# Autodesk Inventor assembly: Shooter assembly
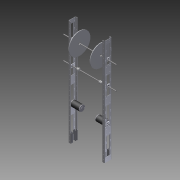
[picture p0: Inventor's stored thumbnail of the model, 180x180]
Saved by Autodesk Inventor 2014 SP1 (Build 180222100, 222)
## iProperties
Created: 2014-02-21
Part Number: Shooter assembly
Document SubType Name: Assembly
Designer: Asif
Author: Asif
## Documents named in this file (9)
- C:\Users\Asif\Documents\GitHub\CAD\CAD Team 2014\Shooter\Shooter assembly.iam
- C:\Users\Asif\Documents\GitHub\CAD\CAD Team 2014\Shooter\U-CHANNEL 6 Sot_sheet metal Edited to size.ipt
- C:\Users\Asif\Documents\GitHub\CAD\CAD Team 2014\Shooter\8020-1010 edited to size.ipt
- C:\Users\Asif\Documents\GitHub\CAD\CAD Team 2014\Shooter\CIM RECEIVER - AM-0860.ipt
- C:\Users\Asif\Documents\GitHub\CAD\CAD Team 2014\Shooter\3-8 bearing.ipt
- C:\Users\Asif\Documents\GitHub\CAD\CAD Team 2014\Shooter\80t Sprocket.ipt
- C:\Users\Asif\Documents\GitHub\CAD\CAD Team 2014\Shooter\3-8 Shooter Shaft.ipt
- C:\Users\Asif\Documents\GitHub\CAD\CAD Team 2014\Shooter\10 th sprocket.ipt
- C:\Users\Asif\Documents\GitHub\CAD\CAD Team 2014\Shooter\CIM motor.ipt
## Components (24 placed, 8 different names)
1. U-CHANNEL 6 Sot_sheet metal Edited to size:1 — Mate:1, Mate:2, Mate:3, Mate:4, Flush:2, Flush:5, Flush:6, Flush:7, Mate:16, Mate:17, Mate:25, Mate:26, Flush:13, Mate:27, Mate:28
2. U-CHANNEL 6 Sot_sheet metal Edited to size:2 — Mate:5, Mate:6, Flush:3, Mate:7, Mate:8, Flush:4, Flush:6, Flush:7, Mate:10, Mate:11, Mate:12, Mate:13, Mate:14, Mate:15, Flush:13
3. 8020-1010 edited to size:1 — Mate:3, Mate:4, Flush:2
4. 8020-1010 edited to size:2 — Mate:1, Mate:2, Flush:5, Tangent:1
5. 8020-1010 edited to size:3 — Mate:5, Mate:6, Flush:3, Tangent:1
6. 8020-1010 edited to size:4 — Mate:7, Mate:8, Flush:4
7. CIM RECEIVER - AM-0860:1 — Insert:8, Flush:9, Mate:25, Mate:26
8. CIM RECEIVER - AM-0860:2 — Mate:14, Mate:15, Insert:4, Flush:8
9. CIM RECEIVER - AM-0860:3 — Mate:10, Mate:11, Insert:7, Flush:9
10. CIM RECEIVER - AM-0860:4 — Mate:12, Mate:13, Flush:10, Insert:14
11. CIM RECEIVER - AM-0860:5 — Flush:10, Insert:13, Mate:27, Mate:28
12. CIM RECEIVER - AM-0860:6 — Mate:16, Mate:17, Insert:1, Flush:8
13. 3-8 bearing:2 — Insert:4, Mate:22, Insert:12
14. 3-8 bearing:3 — Insert:7
15. 3-8 bearing:4 — Insert:1, Mate:21, Insert:9, Insert:11
16. 3-8 bearing:6 — Insert:8, Insert:10
17. 80t Sprocket:1 — Insert:11, Flush:11
18. 80t Sprocket:2 — Insert:12, Flush:12
19. 3-8 Shooter Shaft:1 — Insert:9
20. 3-8 Shooter Shaft:2 — Insert:10, Mate:23, Mate:24
21. 10 th sprocket:1 — Flush:11, Mate:23
22. 10 th sprocket:2 — Flush:12, Mate:24
23. CIM motor:1 — Insert:13
24. CIM motor:2 — Insert:14
## Relationships (47: Mate 24, Flush 12, Insert 10, Tangent 1)
- Mate:1: U-CHANNEL 6 Sot_sheet metal Edited to size:1 ↔ 8020-1010 edited to size:2
- Mate:2: U-CHANNEL 6 Sot_sheet metal Edited to size:1 ↔ 8020-1010 edited to size:2
- Mate:3: U-CHANNEL 6 Sot_sheet metal Edited to size:1 ↔ 8020-1010 edited to size:1
- Mate:4: U-CHANNEL 6 Sot_sheet metal Edited to size:1 ↔ 8020-1010 edited to size:1
- Flush:2: U-CHANNEL 6 Sot_sheet metal Edited to size:1 ↔ 8020-1010 edited to size:1
- Mate:5: U-CHANNEL 6 Sot_sheet metal Edited to size:2 ↔ 8020-1010 edited to size:3
- Mate:6: U-CHANNEL 6 Sot_sheet metal Edited to size:2 ↔ 8020-1010 edited to size:3
- Flush:3: U-CHANNEL 6 Sot_sheet metal Edited to size:2 ↔ 8020-1010 edited to size:3
- Mate:7: U-CHANNEL 6 Sot_sheet metal Edited to size:2 ↔ 8020-1010 edited to size:4
- Mate:8: U-CHANNEL 6 Sot_sheet metal Edited to size:2 ↔ 8020-1010 edited to size:4
- Flush:4: U-CHANNEL 6 Sot_sheet metal Edited to size:2 ↔ 8020-1010 edited to size:4
- Flush:5: U-CHANNEL 6 Sot_sheet metal Edited to size:1 ↔ 8020-1010 edited to size:2
- Flush:6: U-CHANNEL 6 Sot_sheet metal Edited to size:1 ↔ U-CHANNEL 6 Sot_sheet metal Edited to size:2
- Flush:7: U-CHANNEL 6 Sot_sheet metal Edited to size:1 ↔ U-CHANNEL 6 Sot_sheet metal Edited to size:2
- Tangent:1 (381 mm): 8020-1010 edited to size:2 ↔ 8020-1010 edited to size:3
- Mate:10: U-CHANNEL 6 Sot_sheet metal Edited to size:2 ↔ CIM RECEIVER - AM-0860:3
- Mate:11: U-CHANNEL 6 Sot_sheet metal Edited to size:2 ↔ CIM RECEIVER - AM-0860:3
- Mate:12: U-CHANNEL 6 Sot_sheet metal Edited to size:2 ↔ CIM RECEIVER - AM-0860:4
- Mate:13: U-CHANNEL 6 Sot_sheet metal Edited to size:2 ↔ CIM RECEIVER - AM-0860:4
- Mate:14: U-CHANNEL 6 Sot_sheet metal Edited to size:2 ↔ CIM RECEIVER - AM-0860:2
- Mate:15: U-CHANNEL 6 Sot_sheet metal Edited to size:2 ↔ CIM RECEIVER - AM-0860:2
- Mate:16: U-CHANNEL 6 Sot_sheet metal Edited to size:1 ↔ CIM RECEIVER - AM-0860:6
- Mate:17: U-CHANNEL 6 Sot_sheet metal Edited to size:1 ↔ CIM RECEIVER - AM-0860:6
- Insert:1: CIM RECEIVER - AM-0860:6 ↔ 3-8 bearing:4
- Insert:4: CIM RECEIVER - AM-0860:2 ↔ 3-8 bearing:2
- Insert:7: CIM RECEIVER - AM-0860:3 ↔ 3-8 bearing:3
- Insert:8: CIM RECEIVER - AM-0860:1 ↔ 3-8 bearing:6
- Mate:21: 3-8 bearing:4
- Mate:22: 3-8 bearing:2
- Flush:8: CIM RECEIVER - AM-0860:2 ↔ CIM RECEIVER - AM-0860:6
- Flush:9: CIM RECEIVER - AM-0860:1 ↔ CIM RECEIVER - AM-0860:3
- Flush:10: CIM RECEIVER - AM-0860:4 ↔ CIM RECEIVER - AM-0860:5
- Insert:9 (-101.6 mm): 3-8 bearing:4 ↔ 3-8 Shooter Shaft:1
- Insert:10 (-101.6 mm): 3-8 bearing:6 ↔ 3-8 Shooter Shaft:2
- Insert:11 (76.2 mm): 3-8 bearing:4 ↔ 80t Sprocket:1
- Insert:12 (76.2 mm): 3-8 bearing:2 ↔ 80t Sprocket:2
- Flush:11: 80t Sprocket:1 ↔ 10 th sprocket:1
- Mate:23: 3-8 Shooter Shaft:2 ↔ 10 th sprocket:1
- Flush:12: 80t Sprocket:2 ↔ 10 th sprocket:2
- Mate:24: 3-8 Shooter Shaft:2 ↔ 10 th sprocket:2
- Insert:13: CIM RECEIVER - AM-0860:5 ↔ CIM motor:1
- Insert:14: CIM RECEIVER - AM-0860:4 ↔ CIM motor:2
- Mate:25: U-CHANNEL 6 Sot_sheet metal Edited to size:1 ↔ CIM RECEIVER - AM-0860:1
- Mate:26: U-CHANNEL 6 Sot_sheet metal Edited to size:1 ↔ CIM RECEIVER - AM-0860:1
- Flush:13: U-CHANNEL 6 Sot_sheet metal Edited to size:1 ↔ U-CHANNEL 6 Sot_sheet metal Edited to size:2
- Mate:27: U-CHANNEL 6 Sot_sheet metal Edited to size:1 ↔ CIM RECEIVER - AM-0860:5
- Mate:28: U-CHANNEL 6 Sot_sheet metal Edited to size:1 ↔ CIM RECEIVER - AM-0860:5
